# Autodesk Inventor assembly: left drive
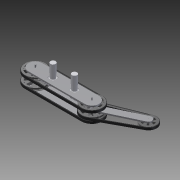
[picture p0: Inventor's stored thumbnail of the model, 180x180]
Saved by Autodesk Inventor 2011 (Build 150239000, 239)
## iProperties
Created: 2010-04-20
Part Number: left drive
Document SubType Name: Assembly
Designer: lucio
Mass: 2596.54 g
Surface Area: 8089.76 cm^2
Volume: 2558.21 cm^3
Density: 1.01499 g/cm^3
Author: lucio
## Documents named in this file (10)
- C:\Users\lucio\Documents\Inventor\caterpillar\left drive.iam
- C:\Users\lucio\Documents\Inventor\caterpillar\base side.ipt
- C:\Users\lucio\Documents\Inventor\caterpillar\mr85vel 2 etapas.ipt
- C:\Users\lucio\Documents\Inventor\caterpillar\mr85vel 3 etapas.ipt
- C:\Users\lucio\Documents\Inventor\caterpillar\back wheel.iam
- C:\Users\lucio\Documents\Inventor\caterpillar\front wheel.iam
- C:\Users\lucio\Documents\Inventor\caterpillar\sprocket.ipt
- C:\Users\lucio\Documents\Inventor\caterpillar\chain.ipt
- C:\Users\lucio\Documents\Inventor\caterpillar\big belt.ipt
- C:\Users\lucio\Documents\Inventor\caterpillar\outer drive side.ipt
## Components (12 placed, 9 different names)
1. base side:1 — Insert:1, Insert:2, Insert:3, Insert:4
2. mr85vel 2 etapas:1 — Insert:1, Flush:2, Mate:2
3. mr85vel 3 etapas:1 — Insert:2, Mate:1, Flush:1
4. back wheel:1 [sub-assembly] — Insert:4, Mate:7, Mate:10, Mate:11, Mate:14
5. front wheel:1 [sub-assembly] — Insert:3, Mate:9, Flush:3, Mate:12, Flush:4, Mate:13, Flush:5
6. sprocket:1 — Mate:1, Flush:1, Mate:3, Mate:4
7. sprocket:2 — Flush:2, Mate:2, Mate:6, Mate:8
8. chain:1 — Mate:3, Mate:4
9. chain:2 — Mate:6, Mate:7, Mate:8
10. big belt:1 — Mate:9, Flush:3, Mate:10
11. big belt:2 — Mate:11, Mate:12, Flush:4
12. outer drive side:1 — Mate:13, Flush:5, Mate:14
## Relationships (22: Mate 13, Flush 5, Insert 4)
- Insert:1: base side:1 ↔ mr85vel 2 etapas:1
- Insert:2: base side:1 ↔ mr85vel 3 etapas:1
- Insert:3 (2 mm): base side:1 ↔ front wheel:1
- Insert:4 (2 mm): base side:1 ↔ back wheel:1
- Mate:1: mr85vel 3 etapas:1 ↔ sprocket:1
- Flush:1: mr85vel 3 etapas:1 ↔ sprocket:1
- Flush:2: mr85vel 2 etapas:1 ↔ sprocket:2
- Mate:2: mr85vel 2 etapas:1 ↔ sprocket:2
- Mate:3 (0.5 mm): sprocket:1 ↔ chain:1
- Mate:4: sprocket:1 ↔ chain:1
- Mate:6: sprocket:2 ↔ chain:2
- Mate:7: back wheel:1 ↔ chain:2
- Mate:8: sprocket:2 ↔ chain:2
- Mate:9: front wheel:1 ↔ big belt:1
- Flush:3 (-2 mm): front wheel:1 ↔ big belt:1
- Mate:10: back wheel:1 ↔ big belt:1
- Mate:11: back wheel:1 ↔ big belt:2
- Mate:12: front wheel:1 ↔ big belt:2
- Flush:4 (2 mm): front wheel:1 ↔ big belt:2
- Mate:13: front wheel:1 ↔ outer drive side:1
- Flush:5: front wheel:1 ↔ outer drive side:1
- Mate:14: back wheel:1 ↔ outer drive side:1
